# Autodesk Inventor assembly: gripper_testing
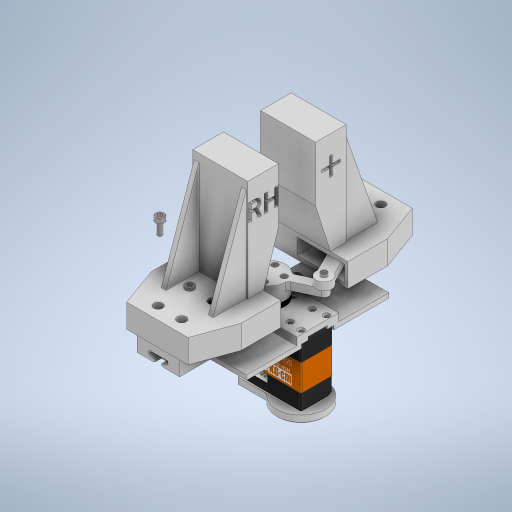
[picture p0: Inventor's stored thumbnail of the model, 512x512]
Saved by Autodesk Inventor 2024 (Build 280153000, 153)
## iProperties
Created: 2023-10-13
Part Number: gripper_testing
Document SubType Name: Assembly
Designer: 박동준
Author: 박동준
## Documents named in this file (14)
- C:\Users\박동준\OneDrive - 연세대학교 (Yonsei University)\바탕 화면\박동준\대학생할\로봇\Humanoid\6축 매니퓰레이터\하드웨어\rh_plus_7_axis_robot_arm_hardware\Assembly\3_Gripper.iam
- C:\Users\박동준\OneDrive - 연세대학교 (Yonsei University)\바탕 화면\박동준\대학생할\로봇\Humanoid\6축 매니퓰레이터\하드웨어\rh_plus_7_axis_robot_arm_hardware\Part\Frame\gripper\gripper.ipt
- C:\Users\박동준\OneDrive - 연세대학교 (Yonsei University)\바탕 화면\박동준\대학생할\로봇\Humanoid\6축 매니퓰레이터\하드웨어\rh_plus_7_axis_robot_arm_hardware\Part\Frame\gripper\gripper_base_frame.ipt
- C:\Users\박동준\OneDrive - 연세대학교 (Yonsei University)\바탕 화면\박동준\대학생할\로봇\Humanoid\6축 매니퓰레이터\하드웨어\rh_plus_7_axis_robot_arm_hardware\Part\Frame\axis_7_top_frame.ipt
- C:\Users\박동준\OneDrive - 연세대학교 (Yonsei University)\바탕 화면\박동준\대학생할\로봇\Humanoid\6축 매니퓰레이터\하드웨어\rh_plus_7_axis_robot_arm_hardware\Part\Frame\gripper\gripper_hand_connector.ipt
- C:\Users\박동준\OneDrive - 연세대학교 (Yonsei University)\바탕 화면\박동준\대학생할\로봇\Humanoid\6축 매니퓰레이터\하드웨어\rh_plus_7_axis_robot_arm_hardware\Part\Other Parts\lm_guide_cart.ipt
- C:\Users\박동준\OneDrive - 연세대학교 (Yonsei University)\바탕 화면\박동준\대학생할\로봇\Humanoid\6축 매니퓰레이터\하드웨어\rh_plus_7_axis_robot_arm_hardware\Part\Other Parts\lm_guide_rail.ipt
- C:\Users\박동준\OneDrive - 연세대학교 (Yonsei University)\바탕 화면\박동준\대학생할\로봇\Humanoid\6축 매니퓰레이터\하드웨어\rh_plus_7_axis_robot_arm_hardware\Part\HTD-45H, Horn\HTD-45H\HTD-45H.iam
- C:\Users\박동준\OneDrive - 연세대학교 (Yonsei University)\바탕 화면\박동준\대학생할\로봇\Humanoid\6축 매니퓰레이터\하드웨어\rh_plus_7_axis_robot_arm_hardware\Part\HTD-45H, Horn\Horn\Top Horn.ipt
- C:\Users\박동준\OneDrive - 연세대학교 (Yonsei University)\바탕 화면\박동준\대학생할\로봇\Humanoid\6축 매니퓰레이터\하드웨어\rh_plus_7_axis_robot_arm_hardware\Part\Bolt, Bearing\m2x10.ipt
- C:\Users\박동준\OneDrive - 연세대학교 (Yonsei University)\바탕 화면\박동준\대학생할\로봇\Humanoid\6축 매니퓰레이터\하드웨어\rh_plus_7_axis_robot_arm_hardware\Part\Bolt, Bearing\m3x8.ipt
- C:\Users\박동준\OneDrive - 연세대학교 (Yonsei University)\바탕 화면\박동준\대학생할\로봇\Humanoid\6축 매니퓰레이터\하드웨어\rh_plus_7_axis_robot_arm_hardware\Part\Frame\axis_7_bottom_frame.ipt
- C:\Users\박동준\OneDrive - 연세대학교 (Yonsei University)\바탕 화면\박동준\대학생할\로봇\Humanoid\6축 매니퓰레이터\하드웨어\rh_plus_7_axis_robot_arm_hardware\Part\Bolt, Bearing\2030 Teflon Sheet.ipt
- C:\Users\박동준\OneDrive - 연세대학교 (Yonsei University)\바탕 화면\박동준\대학생할\로봇\Humanoid\6축 매니퓰레이터\하드웨어\rh_plus_7_axis_robot_arm_hardware\Part\Bolt, Bearing\M2x6 Round Bolt.ipt
## Components (50 placed, 13 different names)
1. 2030 Teflon Sheet:1 — Rigid:12
2. m3x8:12 — Rotational:17
3. m3x8:13
4. m3x8:14 — Rotational:18
5. M2x6 Round Bolt:10 — Rigid:9
6. M2x6 Round Bolt:9 — Rigid:10
7. M2x6 Round Bolt:8 — Rigid:5
8. M2x6 Round Bolt:7 — Rigid:8
9. M2x6 Round Bolt:6 — Rigid:7
10. M2x6 Round Bolt:5 — Rigid:3
11. M2x6 Round Bolt:4 — Rigid:11
12. M2x6 Round Bolt:3 — Rigid:6
13. M2x6 Round Bolt:2 — Rigid:4
14. M2x6 Round Bolt:1 — Rigid:2
15. M2x6 Round Bolt:11 — Rigid:20
16. M2x6 Round Bolt:13 — Rigid:19
17. M2x6 Round Bolt:14 — Rigid:15
18. M2x6 Round Bolt:15 — Rigid:18
19. M2x6 Round Bolt:17 — Rigid:17
20. M2x6 Round Bolt:18 — Rigid:14
21. M2x6 Round Bolt:19 — Rigid:13
22. M2x6 Round Bolt:21 — Rigid:16
23. m2x10:1 — Rotational:1
24. m3x8:1 — Rotational:13
25. m2x10:2 — Rotational:2
26. m2x10:3 — Rotational:4
27. m2x10:4 — Rotational:3
28. m2x10:13 — Mate:45, Mate:46
29. m3x8:2 — Rotational:14
30. m3x8:3 — Rotational:16
31. m3x8:4 — Rotational:15
32. m3x8:9 — Rigid:24
33. m3x8:10 — Rigid:25
34. m3x8:11 — Rigid:26
35. m3x8:8 — Rigid:21
36. m3x8:7 — Rigid:23
37. m3x8:6 — Rigid:22
38. gripper_base_frame:1 — Mate:3, Mate:4, Mate:5, Mate:24, Mate:25, Mate:30, Rotational:1, Rotational:2, Rotational:3, Rotational:4, Mate:43
39. axis_7_top_frame:1 — Mate:10, Mate:11, Angle:1, Mate:12, Mate:13, Mate:14, Mate:15, Mate:16, Mate:17, Rigid:13, Rigid:14, Rigid:15, Rigid:16, Rigid:17, Rigid:18, Rigid:19, Rigid:20
40. axis_7_bottom_frame:1 — Rigid:1, Rigid:2, Rigid:3, Rigid:4, Rigid:5, Rigid:6, Rigid:7, Rigid:8, Rigid:9, Rigid:10, Rigid:11, Rigid:12
41. HTD-45H:1 [sub-assembly] — Mate:1, Mate:2, Mate:10, Mate:11, Angle:1, Mate:49, Flush:2, Flush:3, Rigid:1
42. Top Horn:1 — Mate:1, Mate:2, Mate:3, Mate:4, Mate:5
43. gripper:1 — Angle:4, Flush:1, Mate:44, Rigid:25, Rigid:26, Rigid:24, Mate:50, Mate:51
44. gripper:2 — Mate:26, Mate:27, Angle:5, Mate:28, Flush:1, Rigid:21, Rigid:22, Rigid:23, Mate:52, Rotational:18
45. gripper_hand_connector:1 — Mate:30, Mate:43, Rotational:17, Mate:52
46. gripper_hand_connector:2 — Mate:24, Mate:25, Mate:45, Mate:46, Mate:51
47. lm_guide_cart:1 — Mate:18, Angle:2, Mate:19, Mate:26, Mate:27, Angle:5, Mate:28
48. lm_guide_cart:2 — Mate:20, Angle:3, Mate:21, Angle:4, Mate:44, Mate:50
49. lm_guide_rail:1 — Mate:12, Mate:13, Mate:14, Mate:18, Angle:2, Mate:19, Rotational:13, Rotational:14
50. lm_guide_rail:2 — Mate:15, Mate:16, Mate:17, Mate:20, Angle:3, Mate:21, Rotational:15, Rotational:16
## Relationships (75: Mate 31, WeldJoint 26, RevoluteJoint 10, Angle 5, Flush 3)
- Mate:1: HTD-45H:1 ↔ Top Horn:1
- Mate:2: HTD-45H:1 ↔ Top Horn:1
- Mate:3: gripper_base_frame:1 ↔ Top Horn:1
- Mate:4: gripper_base_frame:1 ↔ Top Horn:1
- Mate:5: gripper_base_frame:1 ↔ Top Horn:1
- Mate:10: axis_7_top_frame:1 ↔ HTD-45H:1
- Mate:11: axis_7_top_frame:1 ↔ HTD-45H:1
- Angle:1 (0 deg): axis_7_top_frame:1 ↔ HTD-45H:1
- Mate:12: axis_7_top_frame:1 ↔ lm_guide_rail:1
- Mate:13: axis_7_top_frame:1 ↔ lm_guide_rail:1
- Mate:14: axis_7_top_frame:1 ↔ lm_guide_rail:1
- Mate:15: axis_7_top_frame:1 ↔ lm_guide_rail:2
- Mate:16: axis_7_top_frame:1 ↔ lm_guide_rail:2
- Mate:17: axis_7_top_frame:1 ↔ lm_guide_rail:2
- Mate:18: lm_guide_cart:1 ↔ lm_guide_rail:1
- Angle:2 (0 deg): lm_guide_cart:1 ↔ lm_guide_rail:1
- Mate:19: lm_guide_cart:1 ↔ lm_guide_rail:1
- Mate:20: lm_guide_cart:2 ↔ lm_guide_rail:2
- Angle:3 (0 deg): lm_guide_cart:2 ↔ lm_guide_rail:2
- Mate:21: lm_guide_cart:2 ↔ lm_guide_rail:2
- Mate:24: gripper_base_frame:1 ↔ gripper_hand_connector:2
- Mate:25: gripper_base_frame:1 ↔ gripper_hand_connector:2
- Angle:4 (0 deg): gripper:1 ↔ lm_guide_cart:2
- Mate:26: gripper:2 ↔ lm_guide_cart:1
- Mate:27: gripper:2 ↔ lm_guide_cart:1
- Angle:5 (0 deg): gripper:2 ↔ lm_guide_cart:1
- Mate:28: gripper:2 ↔ lm_guide_cart:1
- Mate:30: gripper_base_frame:1 ↔ gripper_hand_connector:1
- Flush:1: gripper:1 ↔ gripper:2
- Rotational:1 [RevoluteJoint]: m2x10:1 ↔ gripper_base_frame:1
- Rotational:2 [RevoluteJoint]: m2x10:2 ↔ gripper_base_frame:1
- Rotational:3 [RevoluteJoint]: m2x10:4 ↔ gripper_base_frame:1
- Rotational:4 [RevoluteJoint]: m2x10:3 ↔ gripper_base_frame:1
- Mate:43: gripper_base_frame:1 ↔ gripper_hand_connector:1
- Rotational:13 [RevoluteJoint]: m3x8:1 ↔ lm_guide_rail:1
- Rotational:14 [RevoluteJoint]: m3x8:2 ↔ lm_guide_rail:1
- Rotational:15 [RevoluteJoint]: m3x8:4 ↔ lm_guide_rail:2
- Mate:44: gripper:1 ↔ lm_guide_cart:2
- Rotational:16 [RevoluteJoint]: m3x8:3 ↔ lm_guide_rail:2
- Mate:45: m2x10:13 ↔ gripper_hand_connector:2
- Mate:46: m2x10:13 ↔ gripper_hand_connector:2
- Mate:49: HTD-45H:1
- Flush:2: HTD-45H:1
- Flush:3: HTD-45H:1
- Rigid:1 [WeldJoint]: axis_7_bottom_frame:1 ↔ HTD-45H:1
- Rigid:2 [WeldJoint]: M2x6 Round Bolt:1 ↔ axis_7_bottom_frame:1
- Rigid:3 [WeldJoint]: M2x6 Round Bolt:5 ↔ axis_7_bottom_frame:1
- Rigid:4 [WeldJoint]: M2x6 Round Bolt:2 ↔ axis_7_bottom_frame:1
- Rigid:5 [WeldJoint]: M2x6 Round Bolt:8 ↔ axis_7_bottom_frame:1
- Rigid:6 [WeldJoint]: M2x6 Round Bolt:3 ↔ axis_7_bottom_frame:1
- Rigid:7 [WeldJoint]: M2x6 Round Bolt:6 ↔ axis_7_bottom_frame:1
- Rigid:8 [WeldJoint]: M2x6 Round Bolt:7 ↔ axis_7_bottom_frame:1
- Rigid:9 [WeldJoint]: M2x6 Round Bolt:10 ↔ axis_7_bottom_frame:1
- Rigid:10 [WeldJoint]: M2x6 Round Bolt:9 ↔ axis_7_bottom_frame:1
- Rigid:11 [WeldJoint]: M2x6 Round Bolt:4 ↔ axis_7_bottom_frame:1
- Rigid:12 [WeldJoint]: 2030 Teflon Sheet:1 ↔ axis_7_bottom_frame:1
- Rigid:13 [WeldJoint]: M2x6 Round Bolt:19 ↔ axis_7_top_frame:1
- Rigid:14 [WeldJoint]: M2x6 Round Bolt:18 ↔ axis_7_top_frame:1
- Rigid:15 [WeldJoint]: M2x6 Round Bolt:14 ↔ axis_7_top_frame:1
- Rigid:16 [WeldJoint]: M2x6 Round Bolt:21 ↔ axis_7_top_frame:1
- Rigid:17 [WeldJoint]: M2x6 Round Bolt:17 ↔ axis_7_top_frame:1
- Rigid:18 [WeldJoint]: M2x6 Round Bolt:15 ↔ axis_7_top_frame:1
- Rigid:19 [WeldJoint]: M2x6 Round Bolt:13 ↔ axis_7_top_frame:1
- Rigid:20 [WeldJoint]: M2x6 Round Bolt:11 ↔ axis_7_top_frame:1
- Rigid:21 [WeldJoint]: m3x8:8 ↔ gripper:2
- Rigid:22 [WeldJoint]: m3x8:6 ↔ gripper:2
- Rigid:23 [WeldJoint]: m3x8:7 ↔ gripper:2
- Rigid:25 [WeldJoint]: m3x8:10 ↔ gripper:1
- Rigid:26 [WeldJoint]: m3x8:11 ↔ gripper:1
- Rigid:24 [WeldJoint]: m3x8:9 ↔ gripper:1
- Rotational:17 [RevoluteJoint]: m3x8:12 ↔ gripper_hand_connector:1
- Mate:50: gripper:1 ↔ lm_guide_cart:2
- Mate:51: gripper:1 ↔ gripper_hand_connector:2
- Mate:52: gripper:2 ↔ gripper_hand_connector:1
- Rotational:18 [RevoluteJoint]: m3x8:14 ↔ gripper:2
